# Autodesk Inventor assembly: 37DEncoderAlBlock
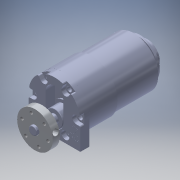
[picture p0: Inventor's stored thumbnail of the model, 180x180]
Saved by Autodesk Inventor 2017 (Build 210142000, 142)
## iProperties
Created: 2017-01-25
Part Number: 37DEncoderAlBlock
Document SubType Name: Assembly
Designer: Naga
Author: Naga
## Documents named in this file (4)
- E:\GDrive\IEEE CS\SoutheastCon2017\Cad\Motors\37DEncoderAlBlock.iam
- E:\GDrive\IEEE CS\SoutheastCon2017\Cad\Brackets\machinedAluminumBracket37dMotor.ipt
- E:\GDrive\IEEE CS\SoutheastCon2017\Cad\Motors\37DEncoder.ipt
- E:\GDrive\IEEE CS\SoutheastCon2017\Cad\Chassis\Wheel Hub.ipt
## Components (3 placed, 3 different names)
1. machinedAluminumBracket37dMotor:1
2. 37DEncoder:1 — Mate:4, Flush:1
3. Wheel Hub:1 — Mate:4, Flush:1
## Relationships (5: Mate 4, Flush 1)
- [Mate]: machinedAluminumBracket37dMotor:1 ↔ 37DEncoder:1
- [Mate]: machinedAluminumBracket37dMotor:1 ↔ 37DEncoder:1
- [Mate]: machinedAluminumBracket37dMotor:1 ↔ 37DEncoder:1
- Mate:4: 37DEncoder:1 ↔ Wheel Hub:1
- Flush:1 (1.5875 mm): 37DEncoder:1 ↔ Wheel Hub:1
## Named parameters: d18_d0 = 0 mm, d19_d1 = 0 mm, d20_d2 = 0 mm
